# Autodesk Inventor assembly: 組合
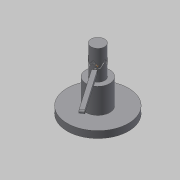
[picture p0: Inventor's stored thumbnail of the model, 180x180]
Saved by Autodesk Inventor 2018 (Build 220112000, 112)
## iProperties
Created: 2021-04-17
Part Number: 組合
Material: 一般
Document SubType Name: Assembly
Designer: 王鼎鈞
Author: 王鼎鈞
## Documents named in this file (5)
- D:\2021顏家民\模組化設計\組合.iam
- D:\2021顏家民\四人圖檔\3d凸輪4-16(第三改法).ipt
- D:\2021顏家民\四人圖檔\支架4-17-2.ipt
- D:\2021顏家民\四人圖檔\主體4-17.ipt
- D:\2021顏家民\四人圖檔\支架4-17縮小球體.ipt
## Components (4 placed, 4 different names)
1. 3d凸輪4-16(第三改法):1 — 插入:1, 旋轉:1, 相切:1, 相切:2
2. 支架4-17-2:1 — 貼合:1, 貼合:2, 貼合:3, 插入:2
3. 主體4-17:1 — 插入:1, 旋轉:1, 插入:2
4. 支架4-17縮小球體:1 — 貼合:1, 貼合:2, 貼合:3, 相切:1, 相切:2
## Relationships (8: Mate 3, Insert 2, Tangent 2, RevoluteJoint 1)
- 插入:1 [Insert]: 3d凸輪4-16(第三改法):1 ↔ 主體4-17:1
- 旋轉:1 [RevoluteJoint]: 3d凸輪4-16(第三改法):1 ↔ 主體4-17:1
- 貼合:1 [Mate] (0.5 mm): 支架4-17-2:1 ↔ 支架4-17縮小球體:1
- 貼合:2 [Mate]: 支架4-17-2:1 ↔ 支架4-17縮小球體:1
- 貼合:3 [Mate]: 支架4-17-2:1 ↔ 支架4-17縮小球體:1
- 插入:2 [Insert]: 支架4-17-2:1 ↔ 主體4-17:1
- 相切:1 [Tangent]: 3d凸輪4-16(第三改法):1 ↔ 支架4-17縮小球體:1
- 相切:2 [Tangent]: 3d凸輪4-16(第三改法):1 ↔ 支架4-17縮小球體:1
